# Autodesk Inventor assembly: Assembly Laser
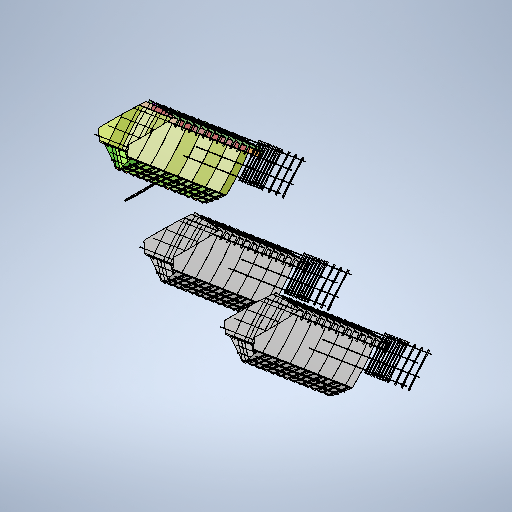
[picture p0: Inventor's stored thumbnail of the model, 512x512]
Saved by Autodesk Inventor 2025 (Build 290162010, 162A)
## iProperties
Created: 2024-09-03
Part Number: Assembly Laser
Document SubType Name: Assembly
Designer: DELL
Author: DELL
## Documents named in this file (6)
- C:\Users\admin\YandexDisk-badmisterfox\домашниий пк\Inventor\Manturovo\Manturovo_Se-clar\DXF файлы\Assembly Laser.iam
- C:\Users\admin\YandexDisk-badmisterfox\домашниий пк\Inventor\Manturovo\Manturovo_Se-clar\ASY MSC 201 BACK.iam
- C:\Users\admin\YandexDisk-badmisterfox\домашниий пк\Inventor\Manturovo\Manturovo_Se-clar\ASY MSC 202 LEFT BOARD.iam
- C:\Users\admin\YandexDisk-badmisterfox\домашниий пк\Inventor\Manturovo\Manturovo_Se-clar\ASY MSC 203 RIGHT BOARD.iam
- C:\Users\admin\YandexDisk-badmisterfox\домашниий пк\Inventor\Manturovo\Manturovo_Se-clar\ASY MSC 204 BELLY.iam
- C:\Users\admin\YandexDisk-badmisterfox\домашниий пк\Inventor\Manturovo\Manturovo_Se-clar\MSC 0512 rib back mould .ipt
## Components (25 placed, 5 different names)
1. ASY MSC 201 BACK:1 [sub-assembly]
2. ASY MSC 202 LEFT BOARD:1 [sub-assembly]
3. ASY MSC 203 RIGHT BOARD:1 [sub-assembly]
4. ASY MSC 204 BELLY:1 [sub-assembly]
5. ASY MSC 201 BACK:2 [sub-assembly]
6. ASY MSC 202 LEFT BOARD:2 [sub-assembly]
7. ASY MSC 203 RIGHT BOARD:2 [sub-assembly]
8. ASY MSC 204 BELLY:2 [sub-assembly]
9. ASY MSC 201 BACK:3 [sub-assembly]
10. ASY MSC 202 LEFT BOARD:3 [sub-assembly]
11. ASY MSC 203 RIGHT BOARD:3 [sub-assembly]
12. ASY MSC 204 BELLY:3 [sub-assembly]
13. MSC 0512 rib back mould :1
14. MSC 0512 rib back mould :2
15. MSC 0512 rib back mould :3
16. MSC 0512 rib back mould :4
17. MSC 0512 rib back mould :5
18. MSC 0512 rib back mould :6
19. MSC 0512 rib back mould :7
20. MSC 0512 rib back mould :8
21. MSC 0512 rib back mould :9
22. MSC 0512 rib back mould :10
23. MSC 0512 rib back mould :11
24. MSC 0512 rib back mould :12
25. MSC 0512 rib back mould :13
## Component patterns: (13 elements, first: MSC 0512 rib back mould :1)
## Relationships (12: Mate 12)
- [Mate]: ASY MSC 201 BACK:1 ↔ ASY MSC 203 RIGHT BOARD:1
- [Mate] (-2860 mm): ASY MSC 201 BACK:1 ↔ ASY MSC 204 BELLY:1
- [Mate]: ASY MSC 203 RIGHT BOARD:1 ↔ ASY MSC 204 BELLY:1
- [Mate] (-25 mm): ASY MSC 203 RIGHT BOARD:1 ↔ ASY MSC 204 BELLY:1
- [Mate]: ASY MSC 201 BACK:2 ↔ ASY MSC 203 RIGHT BOARD:2
- [Mate] (-2860 mm): ASY MSC 201 BACK:2 ↔ ASY MSC 204 BELLY:2
- [Mate]: ASY MSC 203 RIGHT BOARD:2 ↔ ASY MSC 204 BELLY:2
- [Mate] (-25 mm): ASY MSC 203 RIGHT BOARD:2 ↔ ASY MSC 204 BELLY:2
- [Mate]: ASY MSC 201 BACK:3 ↔ ASY MSC 203 RIGHT BOARD:3
- [Mate] (-2860 mm): ASY MSC 201 BACK:3 ↔ ASY MSC 204 BELLY:3
- [Mate]: ASY MSC 203 RIGHT BOARD:3 ↔ ASY MSC 204 BELLY:3
- [Mate] (-25 mm): ASY MSC 203 RIGHT BOARD:3 ↔ ASY MSC 204 BELLY:3
## Named parameters: d4_d873 = -2860 mm, d5_d878 = 0 mm, d6_d879 = -25 mm, d7_d858 = 0 mm, d8_d873 = -2860 mm, d9_d878 = 0 mm, d10_d879 = -25 mm, d11_d858 = 0 mm
